# Autodesk Inventor assembly: V1_Cycloid_Assembly
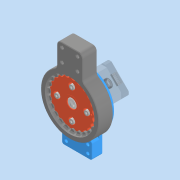
[picture p0: Inventor's stored thumbnail of the model, 180x180]
Saved by Autodesk Inventor 2021 (Build 250183000, 183)
## iProperties
Created: 2020-12-17
Part Number: V1_Cycloid_Assembly
Document SubType Name: Assembly
Designer: ndevr
Author: ndevr
## Documents named in this file (10)
- C:\Sam\Projects\Engineering\DrawBot\DrawBot\Arm\Subsystems\CycoidalDrive - Nema17\V1_N17Cycloid_Assembly.iam
- C:\Sam\Projects\Engineering\DrawBot\DrawBot\Arm\Subsystems\CycoidalDrive - Nema17\Parts\V1_N17Cycloid_RollerBase.ipt
- C:\Sam\Projects\Engineering\DrawBot\DrawBot\Arm\Subsystems\CycoidalDrive - Nema17\Parts\V1_N17Cycloid_CycloidGear.ipt
- C:\Sam\Projects\Engineering\DrawBot\DrawBot\Arm\Subsystems\CycoidalDrive - Nema17\Parts\V1_N17Cycloid_Output.ipt
- C:\Sam\Projects\Engineering\DrawBot\DrawBot\Arm\Subsystems\CycoidalDrive - Nema17\Parts\V1_N17Cycloid_CamShaft.ipt
- C:\Sam\Projects\Engineering\DrawBot\DrawBot\Arm\Subsystems\CycoidalDrive - Nema17\Parts\V1_N17Cycloid_Cam.ipt
- C:\Sam\Projects\Engineering\DrawBot\DrawBot\Arm\Subsystems\CycoidalDrive - Nema17\Geo\V1_N17Cycloid_Geo.ipt
- C:\Sam\Projects\Engineering\DrawBot\DrawBot\Arm\Subsystems\CycoidalDrive - Nema17\Parts\V1_N17Cycloid_AltCam.ipt
- C:\Sam\Projects\Engineering\DrawBot\DrawBot\Arm\Subsystems\CycoidalDrive - Nema17\Parts\V1_N17Cycloid_OutputStandoff.ipt
- C:\Sam\Projects\Engineering\DrawBot\DrawBot\Arm\Subsystems\CycoidalDrive - Nema17\Parts\V1_N17Cycloid_NEMA-17.ipt
## Components (14 placed, 9 different names)
1. V1_N17Cycloid_Geo:1 — Mate:1
2. V1_N17Cycloid_RollerBase:1
3. V1_N17Cycloid_CycloidGear:1
4. V1_N17Cycloid_CycloidGear:2 — Mate:1, Mate:2
5. V1_N17Cycloid_Output:1 — Insert:2, Insert:4, Insert:5, Insert:6, Insert:7, Insert:8, Insert:9
6. V1_N17Cycloid_Output:2 — Insert:8, Insert:9
7. V1_N17Cycloid_CamShaft:1
8. V1_N17Cycloid_Cam:1
9. V1_N17Cycloid_AltCam:1 — Mate:2
10. V1_N17Cycloid_OutputStandoff:1
11. V1_N17Cycloid_OutputStandoff:2 — Insert:5
12. V1_N17Cycloid_OutputStandoff:3 — Insert:6
13. V1_N17Cycloid_OutputStandoff:4 — Insert:2
14. V1_N17Cycloid_NEMA-17:1 — Insert:4, Insert:7
## Relationships (9: Insert 7, Mate 2)
- Mate:1: V1_N17Cycloid_Geo:1 ↔ V1_N17Cycloid_CycloidGear:2
- Mate:2: V1_N17Cycloid_CycloidGear:2 ↔ V1_N17Cycloid_AltCam:1
- Insert:2: V1_N17Cycloid_Output:1 ↔ V1_N17Cycloid_OutputStandoff:4
- Insert:4: V1_N17Cycloid_Output:1 ↔ V1_N17Cycloid_NEMA-17:1
- Insert:5: V1_N17Cycloid_Output:1 ↔ V1_N17Cycloid_OutputStandoff:2
- Insert:6: V1_N17Cycloid_Output:1 ↔ V1_N17Cycloid_OutputStandoff:3
- Insert:7: V1_N17Cycloid_Output:1 ↔ V1_N17Cycloid_NEMA-17:1
- Insert:8: V1_N17Cycloid_Output:1 ↔ V1_N17Cycloid_Output:2
- Insert:9: V1_N17Cycloid_Output:1 ↔ V1_N17Cycloid_Output:2
